# Autodesk Inventor assembly: HCMUTE-CDT23-BTC_ASEMBLY
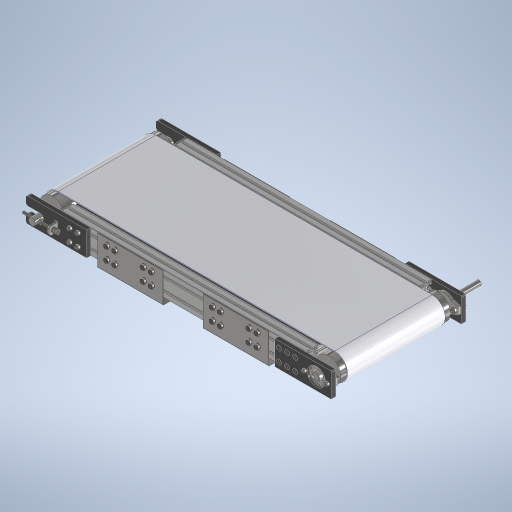
[picture p0: Inventor's stored thumbnail of the model, 512x512]
Saved by Autodesk Inventor 2023 (Build 270158000, 158)
## iProperties
Created: 2023-11-19
Part Number: HCMUTE-CDT23-BTC_ASEMBLY
Document SubType Name: Assembly
Designer: havie
Mass: 19820.2 g
Surface Area: 25718.4 cm^2
Volume: 4225.23 cm^3
Density: 4.69093 g/cm^3
Author: havie
## Documents named in this file (23)
- D:\DO_AN_CDT\1.1. PART\BANG_TAI_CAN\HCMUTE-CDT23-BTC_ASEMBLY.iam
- D:\DO_AN_CDT\1.1. PART\BANG_TAI_CAN\HCMUTE-CDT23-FRAME_BTC_ASEMBLY.iam
- D:\DO_AN_CDT\1.1. PART\BANG_TAI_CAN\HCMUTE-CDT23-BAT_CANG_BANG_TAI.ipt
- D:\DO_AN_CDT\1.1. PART\BANG_TAI_CAN\HCMUTE-CDT23-BAT_TRUC_CANG_TAI.ipt
- D:\DO_AN_CDT\1.1. PART\BANG_TAI_CAN\HCMUTE-CDT23-BAT_TRUC_DAN.ipt
- D:\DO_AN_CDT\1.1. PART\BANG_TAI_CAN\HCMUTE-CDT23-GOI_DO_KFL003.ipt
- D:\DO_AN_CDT\1.1. PART\BANG_TAI_CAN\HCMUTE-CDT23-M6X80_SUOT.ipt
- D:\DO_AN_CDT\1.1. PART\BANG_TAI_CAN\HCMUTE-CDT23-TRUC_CANG.ipt
- D:\DO_AN_CDT\1.1. PART\BANG_TAI_CAN\HCMUTE-CDT23-TRUC_DAN.ipt
- C:\Users\havie\Documents\Inventor\Content Center Files\R2023\en-US\ISO 4762(2)\ISO 4762 - M6 x 16ISO.ipt
- C:\Users\havie\Documents\Inventor\Content Center Files\R2023\en-US\ISO 4762(2)\ISO 4762 - M6 x 25ISO.ipt
- C:\Users\havie\Documents\Inventor\Content Center Files\R2023\en-US\ISO 4032(2)\ISO 4032 - M6 - ISO.ipt
- D:\DO_AN_CDT\1.1. PART\BANG_TAI_CAN\HCMUTE-CDT23-GOI_DO_KFL0031.ipt
- C:\Users\havie\Documents\Inventor\Content Center Files\R2023\en-US\ISO 7092\ISO 7092 - ST 6 - 140 HV.ipt
- D:\DO_AN_CDT\1.1. PART\BANG_TAI_CAN\HCMUTE-CDT23-BAT_CANG_BANG_TAI1.ipt
- D:\DO_AN_CDT\1.1. PART\BANG_TAI_CAN\HCMUTE-CDT23-BAT_TRUC_CANG_TAI1.ipt
- D:\DO_AN_CDT\1.1. PART\BANG_TAI_CAN\HCMUTE-CDT23-M6X80_SUOT1.ipt
- D:\DO_AN_CDT\1.1. PART\BANG_TAI_CAN\HCMUTE-CDT23-BELT_BTC.ipt
- D:\DO_AN_CDT\1.1. PART\BANG_TAI_CAN\HCMUTE-CDT23-MAT_TRUOT.ipt
- C:\Users\havie\Documents\Inventor\Content Center Files\R2023\en-US\ISO 2009(2)\ISO 2009 - M6 x 10 - 4.7 - ISO.ipt
- D:\DO_AN_CDT\1.1. PART\BANG_TAI_CAN\HCMUTE-CDT23-BAT_DO_BTC.ipt
- C:\Users\havie\Documents\Inventor\Content Center Files\R2023\en-US\ISO 4762(2)\ISO 4762 - M6 x 10ISO.ipt
- C:\Users\havie\Documents\Inventor\Content Center Files\R2023\en-US\ISO 4762(2)\ISO 4762 - M6 x 12ISO.ipt
## Components (87 placed, 22 different names)
1. HCMUTE-CDT23-FRAME_BTC_ASEMBLY:1 [sub-assembly] — Mate:1, Flush:1, Flush:2, Mate:25, Flush:5, Mate:26, Mate:27, Mate:28, Mate:68, Mate:69, Flush:6, Mate:70, Mate:75, Flush:7, Mate:77, Flush:8, Mate:87, Tangent:1, Tangent:3
2. HCMUTE-CDT23-BAT_CANG_BANG_TAI:1 — Mate:26, Mate:27, Mate:28, Mate:29, Mate:30, Mate:41, Mate:63
3. HCMUTE-CDT23-BAT_TRUC_CANG_TAI:1 — Mate:25, Flush:5, Mate:29, Mate:31, Mate:32, Mate:33, Mate:34, Mate:35, Mate:36, Mate:37, Mate:38, Mate:61, Mate:95
4. HCMUTE-CDT23-BAT_TRUC_DAN:1 — Mate:1, Flush:1, Flush:2, Mate:2, Mate:3, Mate:4, Mate:5, Mate:11, Mate:12, Mate:13, Mate:14, Mate:90, Mate:91, Mate:92, Mate:93, Mate:94
5. HCMUTE-CDT23-GOI_DO_KFL003:1 — Mate:2, Mate:3, Mate:4, Mate:5, Mate:16, Mate:18, Mate:23, Mate:24
6. HCMUTE-CDT23-M6X80_SUOT:1 — Mate:30, Mate:40, Mate:42, Mate:44, Mate:59, Mate:62
7. HCMUTE-CDT23-BAT_TRUC_DAN:2 — Mate:87, Mate:88, Mate:89
8. ISO 4762 M6 x 25:1 — Mate:11, Mate:14, Mate:15
9. ISO 4762 M6 x 25:2 — Mate:12, Mate:13, Mate:17
10. ISO 4032 M6:1 — Mate:17, Mate:18
11. ISO 4032 M6:2 — Mate:15, Mate:16
12. HCMUTE-CDT23-GOI_DO_KFL0031:1 — Mate:19, Mate:21, Mate:88
13. ISO 4762 M6 x 25:3 — Mate:22, Mate:89
14. ISO 4762 M6 x 25:4 — Mate:20
15. ISO 4032 M6:3 — Mate:19, Mate:20
16. ISO 4032 M6:4 — Mate:21, Mate:22
17. HCMUTE-CDT23-TRUC_DAN:1 — Mate:23, Mate:24, Mate:67
18. ISO 4762 M6 x 16:13 — Mate:33, Mate:36
19. ISO 4762 M6 x 16:15 — Mate:32, Mate:38
20. ISO 4762 M6 x 16:16 — Mate:31, Mate:37
21. ISO 4762 M6 x 16:17 — Mate:34, Mate:35
22. ISO 7092 ST 6 - 140 HV:1 — Mate:40, Mate:41, Mate:43
23. ISO 4032 M6:6 — Mate:42, Mate:43, Mate:44
24. HCMUTE-CDT23-BAT_CANG_BANG_TAI1:1 — Mate:45, Mate:46, Mate:55, Mate:65
25. HCMUTE-CDT23-BAT_TRUC_CANG_TAI1:1 — Mate:45, Mate:47, Mate:49, Mate:51, Mate:53
26. HCMUTE-CDT23-M6X80_SUOT1:1 — Mate:46, Mate:57, Mate:60, Mate:64
27. ISO 4762 M6 x 16:18 — Mate:47
28. ISO 4762 M6 x 16:19 — Mate:49
29. ISO 4762 M6 x 16:20 — Mate:51
30. ISO 4762 M6 x 16:21 — Mate:53
31. ISO 7092 ST 6 - 140 HV:2 — Mate:55, Mate:58
32. ISO 4032 M6:7 — Mate:57, Mate:58
33. HCMUTE-CDT23-TRUC_CANG:1 — Mate:59, Mate:60, Mate:61, Mate:66
34. ISO 4032 M6:8 — Mate:62, Mate:63
35. ISO 4032 M6:9 — Mate:64, Mate:65
36. HCMUTE-CDT23-BELT_BTC:1 — Mate:66, Mate:67, Mate:68
37. HCMUTE-CDT23-MAT_TRUOT:1 — Mate:69, Flush:6, Mate:70, Mate:71, Insert:1, Mate:72, Mate:73, Mate:74, Insert:2, Insert:3, Insert:4
38. ISO 2009 M6 x 10 x 4.7:1 — Mate:71, Insert:1
39. ISO 2009 M6 x 10 x 4.7:2 — Mate:72, Insert:4
40. ISO 2009 M6 x 10 x 4.7:3 — Mate:73, Insert:3
41. ISO 2009 M6 x 10 x 4.7:4 — Mate:74, Insert:2
42. HCMUTE-CDT23-BAT_DO_BTC:1 — Mate:75, Flush:7, Mate:95, Tangent:2, Mate:96, Tangent:4, Mate:97
43. HCMUTE-CDT23-BAT_DO_BTC:2 — Mate:77, Flush:8, Mate:94
44. ISO 4762 M6 x 12:7
45. ISO 4762 M6 x 12:8
46. ISO 4762 M6 x 12:9
47. ISO 4762 M6 x 12:10
48. ISO 4762 M6 x 12:11
49. ISO 4762 M6 x 12:12
50. ISO 4762 M6 x 10:17
51. ISO 4762 M6 x 10:18
52. ISO 4762 M6 x 10:19
53. ISO 4762 M6 x 10:20
54. ISO 4762 M6 x 10:21
55. ISO 4762 M6 x 10:22
56. ISO 4762 M6 x 10:23
57. ISO 4762 M6 x 10:24
58. ISO 4762 M6 x 10:25
59. ISO 4762 M6 x 10:26
60. ISO 4762 M6 x 10:27
61. ISO 4762 M6 x 10:28
62. ISO 4762 M6 x 10:29
63. ISO 4762 M6 x 10:30
64. ISO 4762 M6 x 10:31
65. ISO 4762 M6 x 10:32
66. ISO 4762 M6 x 12:1 — Mate:90, Mate:91
67. ISO 4762 M6 x 12:2 — Mate:92, Mate:93
68. ISO 4762 M6 x 12:3
69. ISO 4762 M6 x 12:4
70. ISO 4762 M6 x 12:5
71. ISO 4762 M6 x 12:6
72. ISO 4762 M6 x 10:1 — Tangent:1, Tangent:2, Mate:96
73. ISO 4762 M6 x 10:2 — Tangent:3, Tangent:4, Mate:97
74. ISO 4762 M6 x 10:3
75. ISO 4762 M6 x 10:4
76. ISO 4762 M6 x 10:5
77. ISO 4762 M6 x 10:6
78. ISO 4762 M6 x 10:7
79. ISO 4762 M6 x 10:8
80. ISO 4762 M6 x 10:9
81. ISO 4762 M6 x 10:10
82. ISO 4762 M6 x 10:11
83. ISO 4762 M6 x 10:12
84. ISO 4762 M6 x 10:13
85. ISO 4762 M6 x 10:14
86. ISO 4762 M6 x 10:15
87. ISO 4762 M6 x 10:16
## Component patterns: (3 elements, first: ISO 4762 M6 x 12:1 + ISO 4762 M6 x 12:2), (2 elements), (2 elements), Component Pattern 10:2 (2 elements), (2 elements, first: ISO 4762 M6 x 10:1 + ISO 4762 M6 x 10:2), Component Pattern 9:2 (2 elements), Component Pattern 9:3 (2 elements), Component Pattern 9:4 (2 elements)
## Relationships (90: Mate 76, Flush 6, Insert 4, Tangent 4)
- Mate:1: HCMUTE-CDT23-FRAME_BTC_ASEMBLY:1 ↔ HCMUTE-CDT23-BAT_TRUC_DAN:1
- Flush:1: HCMUTE-CDT23-FRAME_BTC_ASEMBLY:1 ↔ HCMUTE-CDT23-BAT_TRUC_DAN:1
- Flush:2 (-75 mm): HCMUTE-CDT23-FRAME_BTC_ASEMBLY:1 ↔ HCMUTE-CDT23-BAT_TRUC_DAN:1
- Mate:2: HCMUTE-CDT23-BAT_TRUC_DAN:1 ↔ HCMUTE-CDT23-GOI_DO_KFL003:1
- Mate:3: HCMUTE-CDT23-BAT_TRUC_DAN:1 ↔ HCMUTE-CDT23-GOI_DO_KFL003:1
- Mate:4: HCMUTE-CDT23-BAT_TRUC_DAN:1 ↔ HCMUTE-CDT23-GOI_DO_KFL003:1
- Mate:5: HCMUTE-CDT23-BAT_TRUC_DAN:1 ↔ HCMUTE-CDT23-GOI_DO_KFL003:1
- Mate:11: HCMUTE-CDT23-BAT_TRUC_DAN:1 ↔ ISO 4762 M6 x 25:1
- Mate:12: HCMUTE-CDT23-BAT_TRUC_DAN:1 ↔ ISO 4762 M6 x 25:2
- Mate:13: HCMUTE-CDT23-BAT_TRUC_DAN:1 ↔ ISO 4762 M6 x 25:2
- Mate:14: HCMUTE-CDT23-BAT_TRUC_DAN:1 ↔ ISO 4762 M6 x 25:1
- Mate:15: ISO 4762 M6 x 25:1 ↔ ISO 4032 M6:2
- Mate:16: HCMUTE-CDT23-GOI_DO_KFL003:1 ↔ ISO 4032 M6:2
- Mate:17: ISO 4762 M6 x 25:2 ↔ ISO 4032 M6:1
- Mate:18: HCMUTE-CDT23-GOI_DO_KFL003:1 ↔ ISO 4032 M6:1
- Mate:19: HCMUTE-CDT23-GOI_DO_KFL0031:1 ↔ ISO 4032 M6:3
- Mate:20: ISO 4762 M6 x 25:4 ↔ ISO 4032 M6:3
- Mate:21: HCMUTE-CDT23-GOI_DO_KFL0031:1 ↔ ISO 4032 M6:4
- Mate:22: ISO 4762 M6 x 25:3 ↔ ISO 4032 M6:4
- Mate:23: HCMUTE-CDT23-GOI_DO_KFL003:1 ↔ HCMUTE-CDT23-TRUC_DAN:1
- Mate:24 (13 mm): HCMUTE-CDT23-GOI_DO_KFL003:1 ↔ HCMUTE-CDT23-TRUC_DAN:1
- Mate:25: HCMUTE-CDT23-FRAME_BTC_ASEMBLY:1 ↔ HCMUTE-CDT23-BAT_TRUC_CANG_TAI:1
- Flush:5: HCMUTE-CDT23-FRAME_BTC_ASEMBLY:1 ↔ HCMUTE-CDT23-BAT_TRUC_CANG_TAI:1
- Mate:26: HCMUTE-CDT23-FRAME_BTC_ASEMBLY:1 ↔ HCMUTE-CDT23-BAT_CANG_BANG_TAI:1
- Mate:27: HCMUTE-CDT23-FRAME_BTC_ASEMBLY:1 ↔ HCMUTE-CDT23-BAT_CANG_BANG_TAI:1
- Mate:28: HCMUTE-CDT23-FRAME_BTC_ASEMBLY:1 ↔ HCMUTE-CDT23-BAT_CANG_BANG_TAI:1
- Mate:29: HCMUTE-CDT23-BAT_CANG_BANG_TAI:1 ↔ HCMUTE-CDT23-BAT_TRUC_CANG_TAI:1
- Mate:30: HCMUTE-CDT23-BAT_CANG_BANG_TAI:1 ↔ HCMUTE-CDT23-M6X80_SUOT:1
- Mate:31: HCMUTE-CDT23-BAT_TRUC_CANG_TAI:1 ↔ ISO 4762 M6 x 16:16
- Mate:32: HCMUTE-CDT23-BAT_TRUC_CANG_TAI:1 ↔ ISO 4762 M6 x 16:15
- Mate:33: HCMUTE-CDT23-BAT_TRUC_CANG_TAI:1 ↔ ISO 4762 M6 x 16:13
- Mate:34: HCMUTE-CDT23-BAT_TRUC_CANG_TAI:1 ↔ ISO 4762 M6 x 16:17
- Mate:35: HCMUTE-CDT23-BAT_TRUC_CANG_TAI:1 ↔ ISO 4762 M6 x 16:17
- Mate:36: HCMUTE-CDT23-BAT_TRUC_CANG_TAI:1 ↔ ISO 4762 M6 x 16:13
- Mate:37: HCMUTE-CDT23-BAT_TRUC_CANG_TAI:1 ↔ ISO 4762 M6 x 16:16
- Mate:38: HCMUTE-CDT23-BAT_TRUC_CANG_TAI:1 ↔ ISO 4762 M6 x 16:15
- Mate:40: HCMUTE-CDT23-M6X80_SUOT:1 ↔ ISO 7092 ST 6 - 140 HV:1
- Mate:41: HCMUTE-CDT23-BAT_CANG_BANG_TAI:1 ↔ ISO 7092 ST 6 - 140 HV:1
- Mate:42: HCMUTE-CDT23-M6X80_SUOT:1 ↔ ISO 4032 M6:6
- Mate:43: ISO 7092 ST 6 - 140 HV:1 ↔ ISO 4032 M6:6
- Mate:44: HCMUTE-CDT23-M6X80_SUOT:1 ↔ ISO 4032 M6:6
- Mate:45: HCMUTE-CDT23-BAT_CANG_BANG_TAI1:1 ↔ HCMUTE-CDT23-BAT_TRUC_CANG_TAI1:1
- Mate:46: HCMUTE-CDT23-BAT_CANG_BANG_TAI1:1 ↔ HCMUTE-CDT23-M6X80_SUOT1:1
- Mate:47: HCMUTE-CDT23-BAT_TRUC_CANG_TAI1:1 ↔ ISO 4762 M6 x 16:18
- Mate:49: HCMUTE-CDT23-BAT_TRUC_CANG_TAI1:1 ↔ ISO 4762 M6 x 16:19
- Mate:51: HCMUTE-CDT23-BAT_TRUC_CANG_TAI1:1 ↔ ISO 4762 M6 x 16:20
- Mate:53: HCMUTE-CDT23-BAT_TRUC_CANG_TAI1:1 ↔ ISO 4762 M6 x 16:21
- Mate:55: HCMUTE-CDT23-BAT_CANG_BANG_TAI1:1 ↔ ISO 7092 ST 6 - 140 HV:2
- Mate:57: HCMUTE-CDT23-M6X80_SUOT1:1 ↔ ISO 4032 M6:7
- Mate:58: ISO 7092 ST 6 - 140 HV:2 ↔ ISO 4032 M6:7
- Mate:59: HCMUTE-CDT23-M6X80_SUOT:1 ↔ HCMUTE-CDT23-TRUC_CANG:1
- Mate:60: HCMUTE-CDT23-M6X80_SUOT1:1 ↔ HCMUTE-CDT23-TRUC_CANG:1
- Mate:61: HCMUTE-CDT23-BAT_TRUC_CANG_TAI:1 ↔ HCMUTE-CDT23-TRUC_CANG:1
- Mate:62: HCMUTE-CDT23-M6X80_SUOT:1 ↔ ISO 4032 M6:8
- Mate:63 (24 mm): HCMUTE-CDT23-BAT_CANG_BANG_TAI:1 ↔ ISO 4032 M6:8
- Mate:64: HCMUTE-CDT23-M6X80_SUOT1:1 ↔ ISO 4032 M6:9
- Mate:65 (24 mm): HCMUTE-CDT23-BAT_CANG_BANG_TAI1:1 ↔ ISO 4032 M6:9
- Mate:66: HCMUTE-CDT23-TRUC_CANG:1 ↔ HCMUTE-CDT23-BELT_BTC:1
- Mate:67: HCMUTE-CDT23-TRUC_DAN:1 ↔ HCMUTE-CDT23-BELT_BTC:1
- Mate:68 (5 mm): HCMUTE-CDT23-FRAME_BTC_ASEMBLY:1 ↔ HCMUTE-CDT23-BELT_BTC:1
- Mate:69: HCMUTE-CDT23-FRAME_BTC_ASEMBLY:1 ↔ HCMUTE-CDT23-MAT_TRUOT:1
- Flush:6: HCMUTE-CDT23-FRAME_BTC_ASEMBLY:1 ↔ HCMUTE-CDT23-MAT_TRUOT:1
- Mate:70 (5 mm): HCMUTE-CDT23-FRAME_BTC_ASEMBLY:1 ↔ HCMUTE-CDT23-MAT_TRUOT:1
- Mate:71: HCMUTE-CDT23-MAT_TRUOT:1 ↔ ISO 2009 M6 x 10 x 4.7:1
- Insert:1 (2 mm): HCMUTE-CDT23-MAT_TRUOT:1 ↔ ISO 2009 M6 x 10 x 4.7:1
- Mate:72: HCMUTE-CDT23-MAT_TRUOT:1 ↔ ISO 2009 M6 x 10 x 4.7:2
- Mate:73: HCMUTE-CDT23-MAT_TRUOT:1 ↔ ISO 2009 M6 x 10 x 4.7:3
- Mate:74: HCMUTE-CDT23-MAT_TRUOT:1 ↔ ISO 2009 M6 x 10 x 4.7:4
- Insert:2 (2 mm): HCMUTE-CDT23-MAT_TRUOT:1 ↔ ISO 2009 M6 x 10 x 4.7:4
- Insert:3 (2 mm): HCMUTE-CDT23-MAT_TRUOT:1 ↔ ISO 2009 M6 x 10 x 4.7:3
- Insert:4 (2 mm): HCMUTE-CDT23-MAT_TRUOT:1 ↔ ISO 2009 M6 x 10 x 4.7:2
- Mate:75: HCMUTE-CDT23-FRAME_BTC_ASEMBLY:1 ↔ HCMUTE-CDT23-BAT_DO_BTC:1
- Flush:7 (1.5 mm): HCMUTE-CDT23-FRAME_BTC_ASEMBLY:1 ↔ HCMUTE-CDT23-BAT_DO_BTC:1
- Mate:77: HCMUTE-CDT23-FRAME_BTC_ASEMBLY:1 ↔ HCMUTE-CDT23-BAT_DO_BTC:2
- Flush:8 (1.5 mm): HCMUTE-CDT23-FRAME_BTC_ASEMBLY:1 ↔ HCMUTE-CDT23-BAT_DO_BTC:2
- Mate:87: HCMUTE-CDT23-FRAME_BTC_ASEMBLY:1 ↔ HCMUTE-CDT23-BAT_TRUC_DAN:2
- Mate:88: HCMUTE-CDT23-BAT_TRUC_DAN:2 ↔ HCMUTE-CDT23-GOI_DO_KFL0031:1
- Mate:89: HCMUTE-CDT23-BAT_TRUC_DAN:2 ↔ ISO 4762 M6 x 25:3
- Mate:90: HCMUTE-CDT23-BAT_TRUC_DAN:1 ↔ ISO 4762 M6 x 12:1
- Mate:91: HCMUTE-CDT23-BAT_TRUC_DAN:1 ↔ ISO 4762 M6 x 12:1
- Mate:92: HCMUTE-CDT23-BAT_TRUC_DAN:1 ↔ ISO 4762 M6 x 12:2
- Mate:93: HCMUTE-CDT23-BAT_TRUC_DAN:1 ↔ ISO 4762 M6 x 12:2
- Mate:94 (25 mm): HCMUTE-CDT23-BAT_TRUC_DAN:1 ↔ HCMUTE-CDT23-BAT_DO_BTC:2
- Mate:95 (18 mm): HCMUTE-CDT23-BAT_TRUC_CANG_TAI:1 ↔ HCMUTE-CDT23-BAT_DO_BTC:1
- Tangent:1: HCMUTE-CDT23-FRAME_BTC_ASEMBLY:1 ↔ ISO 4762 M6 x 10:1
- Tangent:2: HCMUTE-CDT23-BAT_DO_BTC:1 ↔ ISO 4762 M6 x 10:1
- Mate:96: HCMUTE-CDT23-BAT_DO_BTC:1 ↔ ISO 4762 M6 x 10:1
- Tangent:3: HCMUTE-CDT23-FRAME_BTC_ASEMBLY:1 ↔ ISO 4762 M6 x 10:2
- Tangent:4: HCMUTE-CDT23-BAT_DO_BTC:1 ↔ ISO 4762 M6 x 10:2
- Mate:97: HCMUTE-CDT23-BAT_DO_BTC:1 ↔ ISO 4762 M6 x 10:2
